# Autodesk Inventor assembly: lift prototype
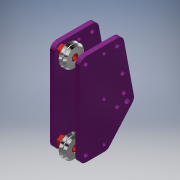
[picture p0: Inventor's stored thumbnail of the model, 180x180]
Saved by Autodesk Inventor 2017 SP1 (Build 210196100, 196)
## iProperties
Created: 2018-01-24
Part Number: lift prototype
Document SubType Name: Assembly
Designer: Ben
Author: Ben
## Documents named in this file (3)
- C:\Users\Ben\Desktop\Projects\2018 Robot\Cube Lift\lift prototype.iam
- C:\Users\Ben\Desktop\Projects\2018 Robot\Cube Lift\carriage plate square 2.ipt
- C:\Users\Ben\Desktop\Projects\2018 Robot\Cube Lift\roller bushing.iam
## Components (5 placed, 2 different names)
1. carriage plate square 2:1 — Insert:2, Insert:3, Insert:4, Mate:1, Mate:2, Mate:3
2. carriage plate square 2:2 — Mate:1, Mate:2, Mate:3
3. roller bushing:1 [sub-assembly] — Insert:4
4. roller bushing:2 [sub-assembly] — Insert:2
5. roller bushing:3 [sub-assembly] — Insert:3
## Relationships (6: Insert 3, Mate 3)
- Insert:2: carriage plate square 2:1 ↔ roller bushing:2
- Insert:3: carriage plate square 2:1 ↔ roller bushing:3
- Insert:4: carriage plate square 2:1 ↔ roller bushing:1
- Mate:1 (30.1244 mm): carriage plate square 2:1 ↔ carriage plate square 2:2
- Mate:2: carriage plate square 2:1 ↔ carriage plate square 2:2
- Mate:3: carriage plate square 2:1 ↔ carriage plate square 2:2
